# Autodesk Inventor assembly: stratos_v2_mechanics
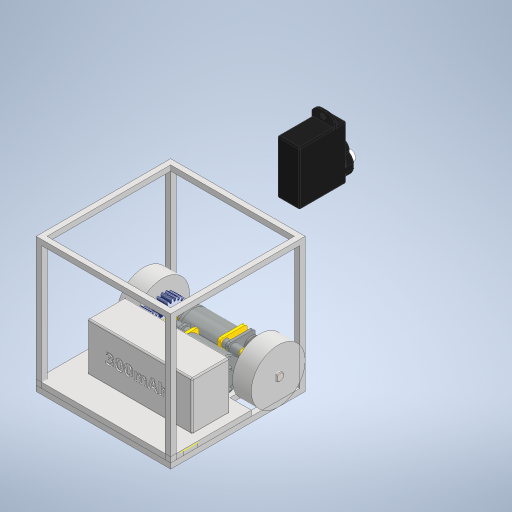
[picture p0: Inventor's stored thumbnail of the model, 512x512]
Saved by Autodesk Inventor 2023.5 (Build 275446000, 446)
## iProperties
Created: 2025-03-17
Part Number: stratos_v2_mechanics
Document SubType Name: Assembly
Designer: kamil
Author: kamil
## Documents named in this file (11)
- E:\PROJECTS_REPOS\Stratos---MicroSumo\mechanics\mechanics V2\stratos_v2_mechanics.iam
- E:\PROJECTS_REPOS\Stratos---MicroSumo\mechanics\Microsumo\mocowanie.ipt
- E:\PROJECTS_REPOS\Stratos---MicroSumo\mechanics\Microsumo\silnik.ipt
- E:\PROJECTS_REPOS\Stratos---MicroSumo\mechanics\Microsumo\zebatka.ipt
- E:\PROJECTS_REPOS\Stratos---MicroSumo\mechanics\mechanics V2\kolo.ipt
- E:\PROJECTS_REPOS\Stratos---MicroSumo\mechanics\mechanics V2\lipo-300.ipt
- E:\PROJECTS_REPOS\Stratos---MicroSumo\mechanics\mechanics V2\MikroSumo\MikroSumo.ipt
- E:\PROJECTS_REPOS\Stratos---MicroSumo\mechanics\mechanics V2\wymiar.ipt
- E:\PROJECTS_REPOS\Stratos---MicroSumo\mechanics\pcb_dolne.ipt
- E:\PROJECTS_REPOS\Stratos---MicroSumo\mechanics\servo_mini_1370hd_cos.ipt
- E:\PROJECTS_REPOS\Stratos---MicroSumo\mechanics\mechanics V2\podstawa_v2.ipt
## Components (13 placed, 10 different names)
1. mocowanie:1 — Zestawiające:2, Kątowe:2, Równoległe:2, Zestawiające:3, Zestawiające:6, Zestawiające:9
2. silnik:1 — Zestawiające:1, Kątowe:1, Równoległe:1, Zestawiające:2, Kątowe:2, Równoległe:3, Zestawiające:5
3. zebatka:1 — Zestawiające:3, Równoległe:4, Zestawiające:8, Zestawiające:9
4. silnik:2 — Zestawiające:1, Kątowe:1, Równoległe:1, Równoległe:2, Równoległe:3, Zestawiające:4, Kątowe:4, Równoległe:9, Zestawiające:14, Zestawiające:17
5. zebatka:2 — Zestawiające:4, Równoległe:4
6. kolo:1 — Zestawiające:5, Zestawiające:7
7. kolo:2 — Zestawiające:6, Zestawiające:7, Zestawiające:8, Równoległe:7, Zestawiające:11, Równoległe:8, Zestawiające:12, Zestawiające:13
8. lipo-300:1 — Równoległe:9, Kątowe:5, Równoległe:18, Zestawiające:17
9. MikroSumo:1 — Równoległe:7, Zestawiające:11, Kątowe:5, Równoległe:10
10. wymiar:1 — Równoległe:8, Zestawiające:12, Zestawiające:13, Kątowe:4, Równoległe:10, Równoległe:11, Równoległe:12, Równoległe:16, Równoległe:17
11. pcb_dolne:1 — Równoległe:11, Równoległe:12
12. servo_mini_1370hd_cos:2
13. podstawa_v2:1 — Zestawiające:14, Równoległe:16, Równoległe:17, Równoległe:18
## Relationships (31: Mate 14, Flush 13, Angle 4)
- Zestawiające:1 [Mate]: silnik:1 ↔ silnik:2
- Kątowe:1 [Angle] (180 deg): silnik:1 ↔ silnik:2
- Równoległe:1 [Flush]: silnik:1 ↔ silnik:2
- Zestawiające:2 [Mate]: mocowanie:1 ↔ silnik:1
- Kątowe:2 [Angle] (0 deg): mocowanie:1 ↔ silnik:1
- Równoległe:2 [Flush] (5 mm): mocowanie:1 ↔ silnik:2
- Równoległe:3 [Flush] (1 mm): silnik:1 ↔ silnik:2
- Zestawiające:3 [Mate]: mocowanie:1 ↔ zebatka:1
- Zestawiające:4 [Mate]: silnik:2 ↔ zebatka:2
- Równoległe:4 [Flush]: zebatka:1 ↔ zebatka:2
- Zestawiające:5 [Mate]: silnik:1 ↔ kolo:1
- Zestawiające:6 [Mate]: mocowanie:1 ↔ kolo:2
- Zestawiające:7 [Mate] (-50 mm): kolo:1 ↔ kolo:2
- Zestawiające:8 [Mate]: zebatka:1 ↔ kolo:2
- Zestawiające:9 [Mate]: mocowanie:1 ↔ zebatka:1
- Równoległe:7 [Flush]: kolo:2 ↔ MikroSumo:1
- Zestawiające:11 [Mate] (15 mm): kolo:2 ↔ MikroSumo:1
- Równoległe:8 [Flush]: kolo:2 ↔ wymiar:1
- Zestawiające:12 [Mate] (-10 mm): kolo:2 ↔ wymiar:1
- Zestawiające:13 [Mate] (-10 mm): kolo:2 ↔ wymiar:1
- Kątowe:4 [Angle] (0 deg): silnik:2 ↔ wymiar:1
- Równoległe:9 [Flush] (1 mm): silnik:2 ↔ lipo-300:1
- Kątowe:5 [Angle] (180 deg): lipo-300:1 ↔ MikroSumo:1
- Równoległe:10 [Flush]: MikroSumo:1 ↔ wymiar:1
- Równoległe:11 [Flush]: wymiar:1 ↔ pcb_dolne:1
- Równoległe:12 [Flush] (-2 mm): wymiar:1 ↔ pcb_dolne:1
- Zestawiające:14 [Mate]: silnik:2 ↔ podstawa_v2:1
- Równoległe:16 [Flush]: wymiar:1 ↔ podstawa_v2:1
- Równoległe:17 [Flush]: wymiar:1 ↔ podstawa_v2:1
- Równoległe:18 [Flush] (2 mm): lipo-300:1 ↔ podstawa_v2:1
- Zestawiające:17 [Mate] (1 mm): silnik:2 ↔ lipo-300:1
